# Autodesk Inventor assembly: Assembly2
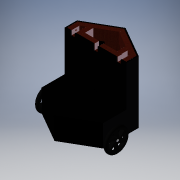
[picture p0: Inventor's stored thumbnail of the model, 180x180]
Saved by Autodesk Inventor 2017 (Build 210142000, 142)
## iProperties
Created: 2018-10-17
Part Number: Assembly2
Document SubType Name: Assembly
Designer: Administrator
Author: Administrator
## Documents named in this file (4)
- C:\Users\Dell\Documents\GitHub\tr2\Base\Base.iam
- C:\Users\Dell\Documents\GitHub\tr2\Base\Base Cover Assembly.iam
- C:\Users\Dell\Documents\GitHub\tr2\Base\Base Chassis Assembly.iam
- C:\Users\Dell\Documents\GitHub\tr2\Wheel Assembly\Wheel Assembly, Right.iam
## Components (4 placed, 3 different names)
1. Base Cover Assembly:1 [sub-assembly] — Mate:124, Mate:125, Mate:126
2. Base Chassis Assembly:1 [sub-assembly] — Mate:121, Mate:123, Flush:3, Mate:124, Mate:125, Mate:126, Mate:127, Flush:4, Flush:5, Mate:128, Mate:130, Mate:131
3. Wheel Assembly, Right:1 [sub-assembly] — Flush:5, Mate:128, Mate:130
4. Wheel Assembly, Right:2 [sub-assembly] — Mate:127, Flush:4, Mate:131
## Relationships (12: Mate 9, Flush 3)
- Mate:121: Base Chassis Assembly:1
- Mate:123: Base Chassis Assembly:1
- Flush:3: Base Chassis Assembly:1
- Mate:124: Base Cover Assembly:1 ↔ Base Chassis Assembly:1
- Mate:125: Base Cover Assembly:1 ↔ Base Chassis Assembly:1
- Mate:126: Base Cover Assembly:1 ↔ Base Chassis Assembly:1
- Mate:127: Base Chassis Assembly:1 ↔ Wheel Assembly, Right:2
- Flush:4: Base Chassis Assembly:1 ↔ Wheel Assembly, Right:2
- Flush:5: Base Chassis Assembly:1 ↔ Wheel Assembly, Right:1
- Mate:128: Base Chassis Assembly:1 ↔ Wheel Assembly, Right:1
- Mate:130: Base Chassis Assembly:1 ↔ Wheel Assembly, Right:1
- Mate:131: Base Chassis Assembly:1 ↔ Wheel Assembly, Right:2
